# Autodesk Inventor assembly: RCT-T003_front_rear_steering_linkage_assembly
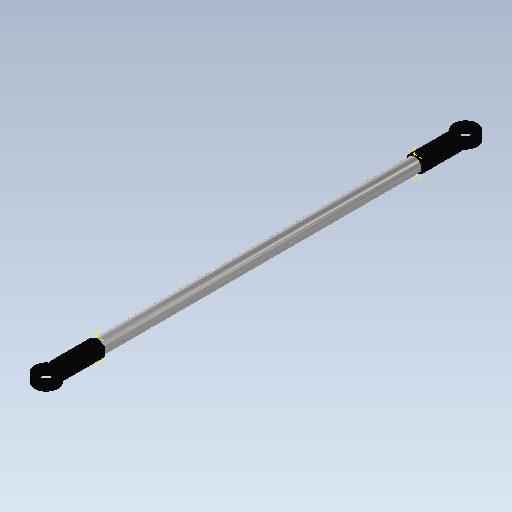
[picture p0: Inventor's stored thumbnail of the model, 512x512]
Saved by Autodesk Inventor 2020 (Build 240168000, 168)
## iProperties
Created: 2019-11-29
Part Number: RCT-T003_front_rear_steering_linkage_assembly
Document SubType Name: Assembly
Designer: maste
Author: maste
## Documents named in this file (3)
- C:\Users\maste\Documents\GitHub\autobot\robot_model\RCT-T003_front_rear_steering_linkage_assembly.iam
- C:\Users\maste\Documents\GitHub\autobot\robot_model\RCT-T003_front_rear_steering_linkage.ipt
- C:\Users\maste\Documents\GitHub\autobot\robot_model\RCT-T003 (2).ipt
## Components (3 placed, 2 different names)
1. RCT-T003_front_rear_steering_linkage:1 — Insert:1, Insert:2
2. RCT-T003 (2):1 — Insert:1, Flush:1
3. RCT-T003 (2):2 — Insert:2, Flush:1
## Relationships (3: Insert 2, Flush 1)
- Insert:1: RCT-T003_front_rear_steering_linkage:1 ↔ RCT-T003 (2):1
- Insert:2: RCT-T003_front_rear_steering_linkage:1 ↔ RCT-T003 (2):2
- Flush:1: RCT-T003 (2):1 ↔ RCT-T003 (2):2
